# Autodesk Inventor assembly: Boss_Assembly
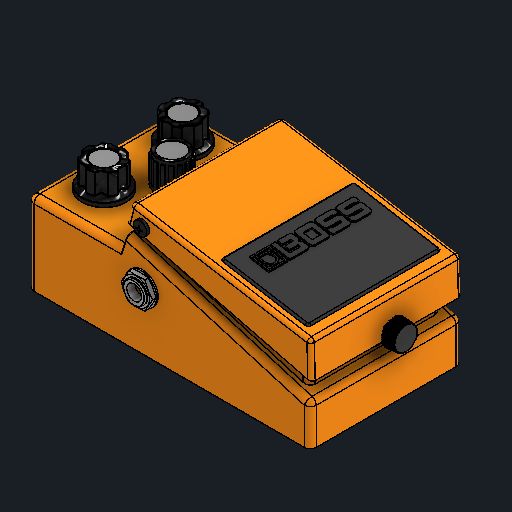
[picture p0: Inventor's stored thumbnail of the model, 512x512]
Saved by Autodesk Inventor 2026.2 (Build 302298000, 298)
## iProperties
Created: 2015-04-29
Part Number: Boss_Assembly
Document SubType Name: Assembly
Designer: Philip
Author: Philip
## Documents named in this file (6)
- C:\Users\JoshuaEah\Documents\GitHub\Designed-Trinkets\Guitar\Modular Pedalboard\Pedals\Boss Pedal\Boss_Assembly.iam
- C:\Users\JoshuaEah\Documents\GitHub\Designed-Trinkets\Guitar\Modular Pedalboard\Pedals\Boss Pedal\Pedal_Assembly.iam
- C:\Users\JoshuaEah\Documents\GitHub\Designed-Trinkets\Guitar\Modular Pedalboard\Pedals\Boss Pedal\Button_Knob.ipt
- C:\Users\JoshuaEah\Documents\GitHub\Designed-Trinkets\Guitar\Modular Pedalboard\Pedals\Boss Pedal\Knob2.ipt
- C:\Users\JoshuaEah\Documents\GitHub\Designed-Trinkets\Guitar\Modular Pedalboard\Pedals\Boss Pedal\Knob3.ipt
- C:\Users\JoshuaEah\Documents\GitHub\Designed-Trinkets\Guitar\Modular Pedalboard\Pedals\Boss Pedal\Frame.iam
## Components (8 placed, 5 different names)
1. Frame:1 [sub-assembly] — Insert:20, Insert:21, Insert:22
2. Pedal_Assembly:1 [sub-assembly]
3. Button_Knob:1 — Insert:17, Insert:20
4. Button_Knob:2 — Insert:18, Insert:22
5. Button_Knob:3 — Insert:19, Insert:21
6. Knob2:1 — Insert:17
7. Knob2:2 — Insert:18
8. Knob3:1 — Insert:19
## Relationships (8: Insert 8)
- Insert:17: Button_Knob:1 ↔ Knob2:1
- Insert:18: Button_Knob:2 ↔ Knob2:2
- Insert:19: Button_Knob:3 ↔ Knob3:1
- Insert:20: Frame:1 ↔ Button_Knob:1
- Insert:21: Frame:1 ↔ Button_Knob:3
- Insert:22: Frame:1 ↔ Button_Knob:2
- [Insert]: Frame:1 ↔ Pedal_Assembly:1
- [Insert]: Frame:1 ↔ Pedal_Assembly:1
